# Autodesk Inventor assembly: Flyspresso-CAD-files:24W SHELL BOTTOM - COVER ONLY
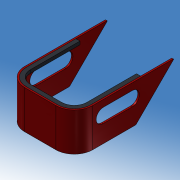
[picture p0: Inventor's stored thumbnail of the model, 180x180]
Saved by Autodesk Inventor 2015 SP1 (Build 190203100, 203)
## iProperties
Created: 2015-07-30
Vendor: HHMI: JRC - ID&F
Document SubType Name: Assembly
Designer: JORDANJ
RuleStatus: InUse
AfterDocSave0: file://Part Number Cleaner
DESIGN DEPARTMENT: HHMI: JRC - ID&F
ALTERED ITEM PART NUMBER: N/A
ALTERED ITEM VENDOR: N/A
ALTERED ITEM DESCRIPTION: N/A
Author: JORDANJ
Revision Number: 0
## Documents named in this file (3)
- C:\_WORKSPACE\DATA\PERSONAL FOLDERS\JORDAN, JEFF\_PROJECTS (SECURE)\LABS & RESEARCH\STERN (LAB)\HYBRIDIZER\MCAD\MICROPLATE\24W SHELL BOTTOM - COVER ONLY.iam
- C:\_WORKSPACE\DATA\PERSONAL FOLDERS\JORDAN, JEFF\_PROJECTS (SECURE)\LABS & RESEARCH\STERN (LAB)\HYBRIDIZER\MCAD\MICROPLATE\24W SHELL BOTTOM.ipt
- C:\_WORKSPACE\DATA\PERSONAL FOLDERS\JORDAN, JEFF\_PROJECTS (SECURE)\LABS & RESEARCH\STERN (LAB)\HYBRIDIZER\MCAD\MICROPLATE\24W SHELL BOTTOM BRACE UPPER.ipt
## Components (2 placed, 2 different names)
1. 24W SHELL BOTTOM:1 — Flush:4, Flush:5, Flush:6
2. 24W SHELL BOTTOM BRACE UPPER:1 — Flush:1, Flush:2, Flush:3
## Relationships (6: Flush 6)
- Flush:1: 24W SHELL BOTTOM BRACE UPPER:1
- Flush:2: 24W SHELL BOTTOM BRACE UPPER:1
- Flush:3: 24W SHELL BOTTOM BRACE UPPER:1
- Flush:4: 24W SHELL BOTTOM:1
- Flush:5: 24W SHELL BOTTOM:1
- Flush:6: 24W SHELL BOTTOM:1
